# Autodesk Inventor assembly: SCR3_15_100A
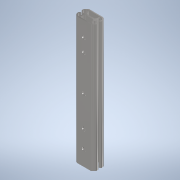
[picture p0: Inventor's stored thumbnail of the model, 180x180]
Saved by Autodesk Inventor 2021 (Build 250183000, 183)
## iProperties
Created: 2014-03-28
Part Number: SCR3_15_100A
Description: STEP AP203
Document SubType Name: Assembly
Designer: Hagihara Yuya
Sending System: SolidWorks 2013
Preprocessor: SwSTEP 2.0
Title: SCR3_15_100A.STEP
Revision Number: ANY
## Documents named in this file (3)
- C:\Users\Hagihara Yuya\Documents\GrabCAD\NHK2021\BasicParts\よく使う部品（萩原）\SlideRail\SlideRail_250\SCR3_15_100A.iam
- C:\Users\Hagihara Yuya\Documents\GrabCAD\NHK2021\BasicParts\よく使う部品（萩原）\SlideRail\SlideRail_250\SCR3_15_100A_outer_SCR3-15-100_.ipt
- C:\Users\Hagihara Yuya\Documents\GrabCAD\NHK2021\BasicParts\よく使う部品（萩原）\SlideRail\SlideRail_250\SCR3_15_100A_inner_SCR3-15-100.ipt
## Components (3 placed, 3 different names)
1. SCR3_15_100A_outer_SCR3-15-100__1 — スライダ:2
2. SCR3_15_100A_outer_SCR3-15-100__2 — スライダ:1
3. SCR3_15_100A_inner_SCR3-15-100_3 — スライダ:1, スライダ:2
## Relationships (2: TranslationJoint 2)
- スライダ:1 [TranslationJoint] (3.45 mm): SCR3_15_100A_outer_SCR3-15-100__2 ↔ SCR3_15_100A_inner_SCR3-15-100_3
- スライダ:2 [TranslationJoint] (3.45 mm): SCR3_15_100A_outer_SCR3-15-100__1 ↔ SCR3_15_100A_inner_SCR3-15-100_3
## Named parameters: Distance1_3 = 3.45 mm, Distance2_3 = 3.45 mm
